# Autodesk Inventor assembly: Alumin Frame
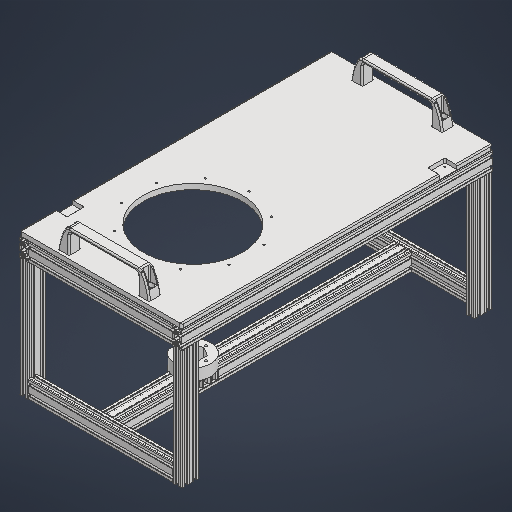
[picture p0: Inventor's stored thumbnail of the model, 512x512]
Saved by Autodesk Inventor 2026.2 (Build 302298000, 298)
## iProperties
Created: 2025-11-19
Part Number: Alumin Frame
Document SubType Name: Assembly
Designer: mumin
Author: mumin
## Documents named in this file (14)
- C:\GitHub\In-situ-monitoring-of-powder-bed-fusion-additive-manufacturing\accessories\Aluminum Test Bench\Aluminum Frame.iam
- C:\GitHub\In-situ-monitoring-of-powder-bed-fusion-additive-manufacturing\accessories\Aluminum Test Bench\4040 Cross Beam (650mm).ipt
- C:\GitHub\In-situ-monitoring-of-powder-bed-fusion-additive-manufacturing\accessories\Aluminum Test Bench\2040 Width Beams (320mm).ipt
- C:\GitHub\In-situ-monitoring-of-powder-bed-fusion-additive-manufacturing\accessories\Aluminum Test Bench\2040 Length Beams (690mm).ipt
- C:\GitHub\In-situ-monitoring-of-powder-bed-fusion-additive-manufacturing\accessories\Aluminum Test Bench\2040 Legs (263.5mm).ipt
- C:\GitHub\In-situ-monitoring-of-powder-bed-fusion-additive-manufacturing\accessories\Aluminum Test Bench\2040 Legs (263.5mm)_MIR.ipt
- C:\GitHub\In-situ-monitoring-of-powder-bed-fusion-additive-manufacturing\accessories\Aluminum Test Bench\2040 Width Beams (320mm)_MIR.ipt
- C:\GitHub\In-situ-monitoring-of-powder-bed-fusion-additive-manufacturing\accessories\Aluminum Test Bench\2040 Legs (263.5mm)_MIR1.ipt
- C:\GitHub\In-situ-monitoring-of-powder-bed-fusion-additive-manufacturing\accessories\Aluminum Test Bench\2040 Legs (263.5mm)_MIR_MIR.ipt
- C:\GitHub\In-situ-monitoring-of-powder-bed-fusion-additive-manufacturing\accessories\Aluminum Test Bench\2040 Length Beams (690mm)_MIR.ipt
- C:\GitHub\In-situ-monitoring-of-powder-bed-fusion-additive-manufacturing\accessories\Aluminum Test Bench\2040 Width Beams (320mm)_MIR1.ipt
- C:\GitHub\In-situ-monitoring-of-powder-bed-fusion-additive-manufacturing\accessories\Aluminum Test Bench\Platform Frame Mount Adapter.ipt
- C:\GitHub\In-situ-monitoring-of-powder-bed-fusion-additive-manufacturing\system_development\Mithril\v0.2\Hardware_design\12mm Cover.ipt
- C:\GitHub\In-situ-monitoring-of-powder-bed-fusion-additive-manufacturing\system_development\Mithril\v0.2\Hardware_design\Handle.ipt
## Components (15 placed, 13 different names)
1. 4040 Cross Beam (650mm):1 — Mate:1, Flush:1, Flush:3, Mate:6, Mate:7
2. 2040 Width Beams (320mm):1 — Mate:1, Flush:1, Flush:3, Mate:2, Flush:4, Flush:5, Flush:14
3. 2040 Legs (263.5mm):1 — Mate:2, Flush:4, Flush:5, Flush:8, Flush:9, Mate:4
4. 2040 Legs (263.5mm)_MIR:1
5. 2040 Width Beams (320mm)_MIR:1 — Flush:6, Flush:7, Mate:3
6. 2040 Legs (263.5mm)_MIR1:1 — Flush:6, Flush:7, Mate:3
7. 2040 Legs (263.5mm)_MIR_MIR:1
8. 2040 Length Beams (690mm):1 — Flush:8, Flush:9, Mate:4, Mate:8, Flush:12, Flush:13
9. 2040 Length Beams (690mm)_MIR:1 — Mate:5, Flush:10, Flush:11
10. 2040 Width Beams (320mm):2 — Mate:5, Flush:10, Flush:11
11. 2040 Width Beams (320mm)_MIR1:1
12. Platform Frame Mount Adapter:1 — Mate:6, Mate:7, Flush:14
13. 12mm Cover:1 — Mate:8, Flush:12, Flush:13, Insert:1, Insert:2
14. Handle:1 — Insert:1
15. Handle:2 — Insert:2
## Relationships (23: Flush 13, Mate 8, Insert 2)
- Mate:1: 4040 Cross Beam (650mm):1 ↔ 2040 Width Beams (320mm):1
- Flush:1: 4040 Cross Beam (650mm):1 ↔ 2040 Width Beams (320mm):1
- Flush:3: 4040 Cross Beam (650mm):1 ↔ 2040 Width Beams (320mm):1
- Mate:2: 2040 Width Beams (320mm):1 ↔ 2040 Legs (263.5mm):1
- Flush:4: 2040 Width Beams (320mm):1 ↔ 2040 Legs (263.5mm):1
- Flush:5: 2040 Width Beams (320mm):1 ↔ 2040 Legs (263.5mm):1
- Flush:6: 2040 Width Beams (320mm)_MIR:1 ↔ 2040 Legs (263.5mm)_MIR1:1
- Flush:7: 2040 Width Beams (320mm)_MIR:1 ↔ 2040 Legs (263.5mm)_MIR1:1
- Mate:3: 2040 Width Beams (320mm)_MIR:1 ↔ 2040 Legs (263.5mm)_MIR1:1
- Flush:8: 2040 Legs (263.5mm):1 ↔ 2040 Length Beams (690mm):1
- Flush:9: 2040 Legs (263.5mm):1 ↔ 2040 Length Beams (690mm):1
- Mate:4: 2040 Legs (263.5mm):1 ↔ 2040 Length Beams (690mm):1
- Mate:5: 2040 Length Beams (690mm)_MIR:1 ↔ 2040 Width Beams (320mm):2
- Flush:10: 2040 Length Beams (690mm)_MIR:1 ↔ 2040 Width Beams (320mm):2
- Flush:11: 2040 Length Beams (690mm)_MIR:1 ↔ 2040 Width Beams (320mm):2
- Mate:6: 4040 Cross Beam (650mm):1 ↔ Platform Frame Mount Adapter:1
- Mate:7: 4040 Cross Beam (650mm):1 ↔ Platform Frame Mount Adapter:1
- Mate:8: 2040 Length Beams (690mm):1 ↔ 12mm Cover:1
- Flush:12: 2040 Length Beams (690mm):1 ↔ 12mm Cover:1
- Flush:13: 2040 Length Beams (690mm):1 ↔ 12mm Cover:1
- Flush:14 (205 mm): 2040 Width Beams (320mm):1 ↔ Platform Frame Mount Adapter:1
- Insert:1: 12mm Cover:1 ↔ Handle:1
- Insert:2: 12mm Cover:1 ↔ Handle:2
